# Autodesk Inventor assembly: arm_MIR
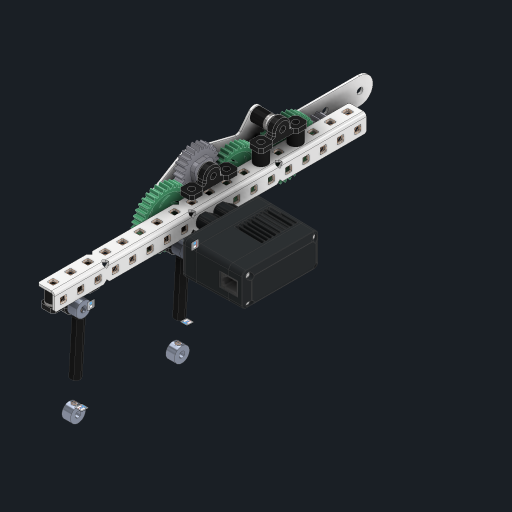
[picture p0: Inventor's stored thumbnail of the model, 512x512]
Saved by Autodesk Inventor 2024 (Build 280153000, 153)
## iProperties
Created: 2023-08-20
Part Number: arm_MIR
Document SubType Name: Assembly
Designer: Averey
Author: Averey
## Documents named in this file (19)
- D:\vex_robotics\hardware\cad\scrap_v0.1\intake\mirrored_parts\arm_MIR.iam
- D:\vex_robotics\hardware\cad\scrap_v0.1\intake\mirrored_parts\Alu Angle 1x1x18_MIR.ipt
- D:\vex_robotics\hardware\cad\VEX-CAD-Inventor-1.41\Motion\Spacers\Spacer Nylon .375 OD\NSpacer .375 OD x .375.ipt
- C:\Users\Averey\Documents\vex\cad\VEX-CAD-Inventor-1.41\Motion\Spacers\Spacer Nylon .375 OD.ipt
- D:\vex_robotics\hardware\cad\scrap_v0.1\intake\mirrored_parts\LS Pillow Bearing Block_MIR.ipt
- D:\vex_robotics\hardware\cad\scrap_v0.1\intake\mirrored_parts\Shaft Collar No Screw_MIR.ipt
- D:\vex_robotics\hardware\cad\VEX-CAD-Inventor-1.41\Motion\Spacers\Washer Steel\SWasher .375 OD x .062500.ipt
- C:\Users\Averey\Documents\vex\cad\VEX-CAD-Inventor-1.41\Motion\Spacers\Washer Steel.ipt
- D:\vex_robotics\hardware\cad\scrap_v0.1\intake\mirrored_parts\LS 36T Gear_MIR.ipt
- D:\vex_robotics\hardware\cad\scrap_v0.1\intake\mirrored_parts\half_cut_24_MIR.ipt
- C:\Users\Averey\Documents\vex\cad\VEX-CAD-Inventor-1.41\Structure\Standoff.ipt
- D:\vex_robotics\hardware\cad\scrap_v0.1\intake\mirrored_parts\V5 Motor (5.5W)_MIR.ipt
- D:\vex_robotics\hardware\cad\scrap_v0.1\intake\custom_parts\intake_gusset.ipt
- D:\vex_robotics\hardware\cad\VEX-CAD-Inventor-1.41\Motion\Shaft LS\LS Pillow Bearing Block.ipt
- D:\vex_robotics\hardware\cad\VEX-CAD-Inventor-1.41\Motion\Spacers\Washer Steel\SWasher .375 OD x .031250.ipt
- D:\vex_robotics\hardware\cad\VEX-CAD-Inventor-1.41\Motion\Spacers\Washer Teflon\TWasher .375 OD x .04000.ipt
- C:\Users\Averey\Documents\vex\cad\VEX-CAD-Inventor-1.41\Motion\Spacers\Washer Teflon.ipt
- D:\vex_robotics\hardware\cad\VEX-CAD-Inventor-1.41\Structure\Standoff\Standoff 1.50.ipt
- D:\vex_robotics\hardware\cad\VEX-CAD-Inventor-1.41\Motion\Gears\LS 12T Gear Steel.ipt
## Components (32 placed, 14 different names)
1. Alu Angle 1x1x18_MIR:1 — Insert:1, Insert:2, Insert:15, Insert:16, Insert:26, Insert:29, Insert:34, Mate:4, Insert:35, Mate:5, Insert:41, Insert:38, Insert:39, Insert:41
2. NSpacer .375 OD x .375:1 — Insert:1, Insert:3
3. NSpacer .375 OD x .375:2 — Insert:2, Insert:4
4. LS Pillow Bearing Block_MIR:1 — Insert:6, Insert:5, Mate:1
5. Shaft Collar No Screw_MIR:1 — Insert:6, Flush:1, Insert:33
6. Shaft Collar No Screw_MIR:2 — Flush:1, Insert:34
7. SWasher .375 OD x .062500:1 — Insert:5, Insert:3
8. SWasher .375 OD x .062500:2 — Mate:1, Insert:4
9. NSpacer .375 OD x .375:3 — Insert:15, Insert:9
10. NSpacer .375 OD x .375:4 — Insert:16, Insert:10
11. LS Pillow Bearing Block_MIR:2 — Insert:12, Insert:11, Mate:2
12. Shaft Collar No Screw_MIR:3 — Insert:12, Flush:2, Insert:36
13. Shaft Collar No Screw_MIR:4 — Flush:2, Insert:35
14. SWasher .375 OD x .062500:3 — Insert:11, Insert:9
15. SWasher .375 OD x .062500:4 — Mate:2, Insert:10
16. LS 36T Gear_MIR:1 — Insert:26, Mate:5
17. LS 36T Gear_MIR:2 — Insert:29
18. LS 36T Gear_MIR:3 — Insert:34, Insert:23
19. LS Pillow Bearing Block_MIR:3 — Mate:4, Insert:35, Insert:36
20. half_cut_24_MIR:1 — Insert:36
21. V5 Motor (5.5W)_MIR:1 — Mate:5, Insert:41
22. intake_gusset:1 — Insert:23, Mate:5
23. LS Pillow Bearing Block:1 — Mate:7, Insert:32, Insert:40, Mate:8
24. NSpacer .375 OD x .375:7
25. SWasher .375 OD x .062500:7
26. SWasher .375 OD x .031250:8 — Mate:7, Insert:32
27. TWasher .375 OD x .04000:1
28. Standoff 1.50:3 — Insert:35, Insert:36
29. Standoff 1.50:4 — Insert:33, Insert:34
30. NSpacer .375 OD x .375:8 — Insert:38, Mate:8
31. NSpacer .375 OD x .375:9 — Insert:39, Insert:40
32. LS 12T Gear Steel:1 — Insert:41
## Relationships (40: Insert 31, Mate 7, Flush 2)
- Insert:1: Alu Angle 1x1x18_MIR:1 ↔ NSpacer .375 OD x .375:1
- Insert:2: Alu Angle 1x1x18_MIR:1 ↔ NSpacer .375 OD x .375:2
- Insert:6: LS Pillow Bearing Block_MIR:1 ↔ Shaft Collar No Screw_MIR:1
- Flush:1: Shaft Collar No Screw_MIR:1 ↔ Shaft Collar No Screw_MIR:2
- Insert:5: LS Pillow Bearing Block_MIR:1 ↔ SWasher .375 OD x .062500:1
- Insert:3: NSpacer .375 OD x .375:1 ↔ SWasher .375 OD x .062500:1
- Mate:1: LS Pillow Bearing Block_MIR:1 ↔ SWasher .375 OD x .062500:2
- Insert:4: NSpacer .375 OD x .375:2 ↔ SWasher .375 OD x .062500:2
- Insert:15: Alu Angle 1x1x18_MIR:1 ↔ NSpacer .375 OD x .375:3
- Insert:16: Alu Angle 1x1x18_MIR:1 ↔ NSpacer .375 OD x .375:4
- Insert:12: LS Pillow Bearing Block_MIR:2 ↔ Shaft Collar No Screw_MIR:3
- Flush:2: Shaft Collar No Screw_MIR:3 ↔ Shaft Collar No Screw_MIR:4
- Insert:11: LS Pillow Bearing Block_MIR:2 ↔ SWasher .375 OD x .062500:3
- Insert:9: NSpacer .375 OD x .375:3 ↔ SWasher .375 OD x .062500:3
- Mate:2: LS Pillow Bearing Block_MIR:2 ↔ SWasher .375 OD x .062500:4
- Insert:10: NSpacer .375 OD x .375:4 ↔ SWasher .375 OD x .062500:4
- Insert:26 (9.9219 mm): Alu Angle 1x1x18_MIR:1 ↔ LS 36T Gear_MIR:1
- Insert:29 (9.9219 mm): Alu Angle 1x1x18_MIR:1 ↔ LS 36T Gear_MIR:2
- Insert:34 (9.9219 mm): Alu Angle 1x1x18_MIR:1 ↔ LS 36T Gear_MIR:3
- Mate:4: Alu Angle 1x1x18_MIR:1 ↔ LS Pillow Bearing Block_MIR:3
- Insert:35 (5.1594 mm): Alu Angle 1x1x18_MIR:1 ↔ LS Pillow Bearing Block_MIR:3
- Insert:36: LS Pillow Bearing Block_MIR:3 ↔ half_cut_24_MIR:1
- Mate:5: Alu Angle 1x1x18_MIR:1 ↔ V5 Motor (5.5W)_MIR:1
- Insert:41: Alu Angle 1x1x18_MIR:1 ↔ V5 Motor (5.5W)_MIR:1
- Insert:23 (2.7781 mm): LS 36T Gear_MIR:3 ↔ intake_gusset:1
- Mate:5: LS 36T Gear_MIR:1 ↔ intake_gusset:1
- [Insert]: SWasher .375 OD x .062500:7 ↔ TWasher .375 OD x .04000:1
- [Insert]: SWasher .375 OD x .031250:8 ↔ TWasher .375 OD x .04000:1
- [Insert]: NSpacer .375 OD x .375:7 ↔ SWasher .375 OD x .062500:7
- Mate:7: LS Pillow Bearing Block:1 ↔ SWasher .375 OD x .031250:8
- Insert:32: LS Pillow Bearing Block:1 ↔ SWasher .375 OD x .031250:8
- Insert:33: Shaft Collar No Screw_MIR:1 ↔ Standoff 1.50:4
- Insert:34 (15.875 mm): Shaft Collar No Screw_MIR:2 ↔ Standoff 1.50:4
- Insert:35 (15.875 mm): Shaft Collar No Screw_MIR:4 ↔ Standoff 1.50:3
- Insert:36: Shaft Collar No Screw_MIR:3 ↔ Standoff 1.50:3
- Insert:38: Alu Angle 1x1x18_MIR:1 ↔ NSpacer .375 OD x .375:8
- Insert:39: Alu Angle 1x1x18_MIR:1 ↔ NSpacer .375 OD x .375:9
- Insert:40: LS Pillow Bearing Block:1 ↔ NSpacer .375 OD x .375:9
- Mate:8: LS Pillow Bearing Block:1 ↔ NSpacer .375 OD x .375:8
- Insert:41 (9.9219 mm): Alu Angle 1x1x18_MIR:1 ↔ LS 12T Gear Steel:1
